(part 1 of 2)
# Autodesk Inventor assembly: 110033226_iam_02_造型房屋一
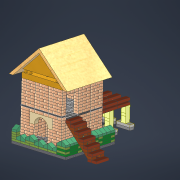
[picture p0: Inventor's stored thumbnail of the model, 180x180]
Saved by Autodesk Inventor 2022 (Build 260153000, 153)
## iProperties
Created: 2022-06-22
Part Number: 110033226_iam_02_造型房屋一
Document SubType Name: Assembly
Designer: User
Author: User
## Documents named in this file (14)
- D:\D-disk\pomelo\大一\下學期\機械設計製圖\1100332260_LEGOproj_沒有公主城堡\110033226_iam_02_造型房屋一.iam
- D:\D-disk\pomelo\大一\下學期\機械設計製圖\1100332260_LEGOproj_沒有公主城堡\110033226_ipt_05_房子底座.ipt
- D:\D-disk\pomelo\大一\下學期\機械設計製圖\1100332260_LEGOproj_沒有公主城堡\110033226_ipt_06_磚塊樺木(1x1).ipt
- D:\D-disk\pomelo\大一\下學期\機械設計製圖\1100332260_LEGOproj_沒有公主城堡\110033226_ipt_07_磚塊樺木(2x1).ipt
- D:\D-disk\pomelo\大一\下學期\機械設計製圖\1100332260_LEGOproj_沒有公主城堡\110033226_ipt_08_平滑面(3x1).ipt
- D:\D-disk\pomelo\大一\下學期\機械設計製圖\1100332260_LEGOproj_沒有公主城堡\110033226_ipt_09_窗戶圓拱.ipt
- D:\D-disk\pomelo\大一\下學期\機械設計製圖\1100332260_LEGOproj_沒有公主城堡\110033226_ipt_02_草地一.ipt
- D:\D-disk\pomelo\大一\下學期\機械設計製圖\1100332260_LEGOproj_沒有公主城堡\110033226_ipt_10_木板條.ipt
- D:\D-disk\pomelo\大一\下學期\機械設計製圖\1100332260_LEGOproj_沒有公主城堡\110033226_ipt_11_樓梯支架.ipt
- D:\D-disk\pomelo\大一\下學期\機械設計製圖\1100332260_LEGOproj_沒有公主城堡\110033226_ipt_12_平滑面(2x1).ipt
- D:\D-disk\pomelo\大一\下學期\機械設計製圖\1100332260_LEGOproj_沒有公主城堡\110033226_ipt_13_草地二.ipt
- D:\D-disk\pomelo\大一\下學期\機械設計製圖\1100332260_LEGOproj_沒有公主城堡\110033226_ipt_14_草地三.ipt
- D:\D-disk\pomelo\大一\下學期\機械設計製圖\1100332260_LEGOproj_沒有公主城堡\110033226_ipt_15_房子屋頂.ipt
- D:\D-disk\pomelo\大一\下學期\機械設計製圖\1100332260_LEGOproj_沒有公主城堡\110033226_ipt_24_直條(3x1).ipt
## Components (694 placed, 13 different names)
1. 110033226_ipt_05_房子底座:1 — 貼合:1, 貼合:2, 貼合:3, 貼合:4, 貼合:6, 貼合:8, 貼合:9, 貼合:10, 貼合:11, 貼合:12, 貼合:13, 貼合:14, 貼合:15, 貼合:16, 貼合:17, 貼合:18, 貼合:19, 貼合:20, 貼合:21, 貼合:22, 貼合:23, 貼合:24, 貼合:25, 貼合:26, 貼合:27, 貼合:28, 貼合:173, 貼合:292, 貼合:293, 貼合:294, 貼合:295, 貼合:296, 貼合:297, 貼合:298, 貼合:299, 貼合:300, 貼合:301, 貼合:302, 貼合:303, 貼合:310, 貼合:311, 貼合:312
2. 110033226_ipt_06_磚塊樺木(1x1):22 — 貼合:37, 貼合:38, 貼合:58, 貼合:59, 貼合:69
3. 110033226_ipt_07_磚塊樺木(2x1):23 — 貼合:34, 貼合:35, 貼合:36, 貼合:60, 貼合:61, 貼合:62
4. 110033226_ipt_06_磚塊樺木(1x1):24 — 貼合:41, 貼合:42, 貼合:68
5. 110033226_ipt_07_磚塊樺木(2x1):25 — 貼合:39, 貼合:40, 貼合:68
6. 110033226_ipt_08_平滑面(3x1):3 — 貼合:93, 貼合:94, 貼合:95
7. 110033226_ipt_09_窗戶圓拱:1 — 貼合:117, 貼合:118, 貼合:119, 貼合:152
8. 110033226_ipt_10_木板條:2 — 貼合:171, 貼合:172, 貼合:173, 貼合:174, 貼合:175, 貼合:176
9. 110033226_ipt_10_木板條:3 — 貼合:177, 貼合:178, 貼合:179
10. 110033226_ipt_10_木板條:4 — 貼合:182, 貼合:186, 貼合:187
11. 110033226_ipt_10_木板條:5 — 貼合:181, 貼合:184, 貼合:185
12. 110033226_ipt_10_木板條:6 — 貼合:183, 貼合:188, 貼合:189
13. 110033226_ipt_10_木板條:7 — 貼合:180, 貼合:190, 貼合:191
14. 110033226_ipt_07_磚塊樺木(2x1):234
15. 110033226_ipt_06_磚塊樺木(1x1):216
16. 110033226_ipt_07_磚塊樺木(2x1):233
17. 110033226_ipt_06_磚塊樺木(1x1):215
18. 110033226_ipt_06_磚塊樺木(1x1):239 — 貼合:246, 貼合:247, 貼合:248, 貼合:264
19. 110033226_ipt_07_磚塊樺木(2x1):257 — 貼合:240, 貼合:241, 貼合:242, 貼合:243, 貼合:244, 貼合:245, 貼合:262
20. 110033226_ipt_06_磚塊樺木(1x1):240 — 貼合:243, 貼合:244, 貼合:245, 貼合:246, 貼合:247, 貼合:248, 貼合:261, 貼合:263
21. 110033226_ipt_07_磚塊樺木(2x1):260 — 貼合:261, 貼合:262, 貼合:263, 貼合:266
22. 110033226_ipt_06_磚塊樺木(1x1):249 — 貼合:264, 貼合:265, 貼合:266
23. 110033226_ipt_06_磚塊樺木(1x1):272
24. 110033226_ipt_08_平滑面(3x1):34 — 貼合:286, 貼合:287, 貼合:288, 貼合:291
25. 110033226_ipt_08_平滑面(3x1):35 — 貼合:283, 貼合:284, 貼合:285
26. 110033226_ipt_12_平滑面(2x1):1 — 貼合:289, 貼合:290, 貼合:291
27. 110033226_ipt_14_草地三:2 — 貼合:307, 貼合:308, 貼合:309, 貼合:315, 貼合:320
28. 110033226_ipt_14_草地三:3 — 貼合:313, 貼合:314, 貼合:315
29. 110033226_ipt_14_草地三:4 — 貼合:319, 貼合:320, 貼合:321, 貼合:338
30. 110033226_ipt_13_草地二:20 — 貼合:331, 貼合:332, 貼合:333, 貼合:334, 貼合:335, 對稱:4, 貼合:369, 貼合:370, 貼合:396
31. 110033226_ipt_13_草地二:21 — 貼合:356, 貼合:357, 貼合:358, 貼合:361, 貼合:363, 貼合:364, 貼合:392, 貼合:393
32. 110033226_ipt_13_草地二:22 — 貼合:339, 貼合:340, 貼合:341, 貼合:343, 貼合:383, 貼合:384, 貼合:385, 貼合:386, 貼合:387
33. 110033226_ipt_13_草地二:23 — 貼合:353, 貼合:354, 貼合:355, 貼合:356, 貼合:357, 貼合:358
34. 110033226_ipt_14_草地三:5 — 貼合:336, 貼合:337, 貼合:338
35. 110033226_ipt_14_草地三:6 — 貼合:325, 貼合:326, 貼合:327, 貼合:329
36. 110033226_ipt_14_草地三:7 — 貼合:334, 貼合:335, 對稱:4, 貼合:368
37. 110033226_ipt_14_草地三:8 — 貼合:322, 貼合:323, 貼合:324, 貼合:367
38. 110033226_ipt_14_草地三:9 — 貼合:328, 貼合:329, 貼合:330
39. 110033226_ipt_14_草地三:10 — 貼合:344, 貼合:345, 貼合:346, 貼合:349
40. 110033226_ipt_14_草地三:11 — 貼合:350, 貼合:351, 貼合:352
41. 110033226_ipt_14_草地三:12 — 貼合:342, 貼合:343, 貼合:346
42. 110033226_ipt_14_草地三:13 — 貼合:347, 貼合:348, 貼合:349, 貼合:352
43. 110033226_ipt_14_草地三:14 — 貼合:361, 貼合:363, 貼合:364
44. 110033226_ipt_14_草地三:16 — 貼合:365, 貼合:366, 貼合:367, 貼合:390
45. 110033226_ipt_14_草地三:17 — 貼合:368, 貼合:369, 貼合:370
46. 110033226_ipt_14_草地三:42 — 貼合:383, 貼合:384, 貼合:385, 貼合:388
47. 110033226_ipt_14_草地三:43 — 貼合:386, 貼合:387, 貼合:388
48. 110033226_ipt_14_草地三:44 — 貼合:389, 貼合:390, 貼合:391
49. 110033226_ipt_14_草地三:45 — 貼合:397, 貼合:398, 貼合:399
50. 110033226_ipt_14_草地三:46 — 貼合:394, 貼合:395, 貼合:396, 貼合:398
51. 110033226_ipt_14_草地三:47 — 貼合:392, 貼合:393
52. 110033226_ipt_15_房子屋頂:1 — 貼合:400, 貼合:401, 貼合:402
53. 110033226_ipt_07_磚塊樺木(2x1):1 — 貼合:4, 貼合:8, 貼合:10, 貼合:29, 貼合:30, 貼合:31, 貼合:32
54. 110033226_ipt_06_磚塊樺木(1x1):1 — 貼合:6, 貼合:9, 貼合:33
55. 110033226_ipt_07_磚塊樺木(2x1):3
56. 110033226_ipt_06_磚塊樺木(1x1):3
57. 110033226_ipt_07_磚塊樺木(2x1):4
58. 110033226_ipt_06_磚塊樺木(1x1):4
59. 110033226_ipt_06_磚塊樺木(1x1):2 — 貼合:11, 貼合:13, 貼合:43, 貼合:45
60. 110033226_ipt_07_磚塊樺木(2x1):2 — 貼合:12, 貼合:14, 貼合:15, 貼合:44, 貼合:46, 貼合:47
61. 110033226_ipt_06_磚塊樺木(1x1):5
62. 110033226_ipt_07_磚塊樺木(2x1):5
63. 110033226_ipt_06_磚塊樺木(1x1):6
64. 110033226_ipt_07_磚塊樺木(2x1):6
65. 110033226_ipt_06_磚塊樺木(1x1):7
66. 110033226_ipt_07_磚塊樺木(2x1):7
67. 110033226_ipt_06_磚塊樺木(1x1):8
68. 110033226_ipt_07_磚塊樺木(2x1):8
69. 110033226_ipt_06_磚塊樺木(1x1):9
70. 110033226_ipt_07_磚塊樺木(2x1):9
71. 110033226_ipt_07_磚塊樺木(2x1):10 — 貼合:17, 貼合:18, 貼合:19, 貼合:49, 貼合:54, 貼合:55
72. 110033226_ipt_06_磚塊樺木(1x1):10 — 貼合:16, 貼合:20, 貼合:48, 貼合:50
73. 110033226_ipt_07_磚塊樺木(2x1):11
74. 110033226_ipt_06_磚塊樺木(1x1):11
75. 110033226_ipt_07_磚塊樺木(2x1):12
76. 110033226_ipt_06_磚塊樺木(1x1):12
77. 110033226_ipt_07_磚塊樺木(2x1):13
78. 110033226_ipt_06_磚塊樺木(1x1):13
79. 110033226_ipt_07_磚塊樺木(2x1):14
80. 110033226_ipt_06_磚塊樺木(1x1):14
81. 110033226_ipt_07_磚塊樺木(2x1):15
82. 110033226_ipt_06_磚塊樺木(1x1):15
83. 110033226_ipt_06_磚塊樺木(1x1):17 — 貼合:30, 貼合:31, 貼合:34, 貼合:35, 貼合:70
84. 110033226_ipt_07_磚塊樺木(2x1):18 — 貼合:29, 貼合:32, 貼合:33, 貼合:36, 貼合:37, 貼合:38, 貼合:70
85. 110033226_ipt_06_磚塊樺木(1x1):18 — 貼合:69, 貼合:95
86. 110033226_ipt_07_磚塊樺木(2x1):19 — 貼合:93, 貼合:94
87. 110033226_ipt_06_磚塊樺木(1x1):19 — 貼合:39, 貼合:40
88. 110033226_ipt_07_磚塊樺木(2x1):20 — 貼合:41, 貼合:42
89. 110033226_ipt_07_磚塊樺木(2x1):21 — 貼合:43, 貼合:45, 貼合:46, 貼合:53, 貼合:56, 貼合:57
90. 110033226_ipt_06_磚塊樺木(1x1):25 — 貼合:44, 貼合:47, 貼合:51, 貼合:52
91. 110033226_ipt_07_磚塊樺木(2x1):27
92. 110033226_ipt_06_磚塊樺木(1x1):26
93. 110033226_ipt_07_磚塊樺木(2x1):28
94. 110033226_ipt_06_磚塊樺木(1x1):27
95. 110033226_ipt_07_磚塊樺木(2x1):29
96. 110033226_ipt_06_磚塊樺木(1x1):28
97. 110033226_ipt_07_磚塊樺木(2x1):30
98. 110033226_ipt_06_磚塊樺木(1x1):29
99. 110033226_ipt_07_磚塊樺木(2x1):31
100. 110033226_ipt_06_磚塊樺木(1x1):30
101. 110033226_ipt_06_磚塊樺木(1x1):20 — 貼合:54, 貼合:55, 貼合:63, 貼合:64
102. 110033226_ipt_07_磚塊樺木(2x1):22 — 貼合:48, 貼合:49, 貼合:50, 貼合:65, 貼合:66, 貼合:67
103. 110033226_ipt_06_磚塊樺木(1x1):31
104. 110033226_ipt_07_磚塊樺木(2x1):32
105. 110033226_ipt_06_磚塊樺木(1x1):32
106. 110033226_ipt_07_磚塊樺木(2x1):33
107. 110033226_ipt_06_磚塊樺木(1x1):33
108. 110033226_ipt_07_磚塊樺木(2x1):34
109. 110033226_ipt_06_磚塊樺木(1x1):34
110. 110033226_ipt_07_磚塊樺木(2x1):35
111. 110033226_ipt_06_磚塊樺木(1x1):35
112. 110033226_ipt_07_磚塊樺木(2x1):36
113. 110033226_ipt_06_磚塊樺木(1x1):43 — 貼合:66, 貼合:67, 貼合:72, 貼合:77
114. 110033226_ipt_07_磚塊樺木(2x1):46 — 貼合:63, 貼合:64, 貼合:65, 貼合:72, 貼合:73, 貼合:74, 貼合:75, 貼合:76
115. 110033226_ipt_06_磚塊樺木(1x1):52
116. 110033226_ipt_07_磚塊樺木(2x1):53
117. 110033226_ipt_06_磚塊樺木(1x1):53
118. 110033226_ipt_07_磚塊樺木(2x1):54
119. 110033226_ipt_06_磚塊樺木(1x1):54
120. 110033226_ipt_07_磚塊樺木(2x1):55
121. 110033226_ipt_06_磚塊樺木(1x1):55
122. 110033226_ipt_07_磚塊樺木(2x1):56
123. 110033226_ipt_06_磚塊樺木(1x1):56
124. 110033226_ipt_07_磚塊樺木(2x1):57
125. 110033226_ipt_07_磚塊樺木(2x1):44 — 貼合:75, 貼合:76, 貼合:77, 貼合:78, 貼合:80, 貼合:82, 貼合:83
126. 110033226_ipt_06_磚塊樺木(1x1):42 — 貼合:73, 貼合:74, 貼合:78, 貼合:79, 貼合:81
127. 110033226_ipt_07_磚塊樺木(2x1):58
128. 110033226_ipt_06_磚塊樺木(1x1):57
129. 110033226_ipt_07_磚塊樺木(2x1):59
130. 110033226_ipt_06_磚塊樺木(1x1):58
131. 110033226_ipt_07_磚塊樺木(2x1):60
132. 110033226_ipt_06_磚塊樺木(1x1):59
133. 110033226_ipt_07_磚塊樺木(2x1):61
134. 110033226_ipt_06_磚塊樺木(1x1):60
135. 110033226_ipt_07_磚塊樺木(2x1):62
136. 110033226_ipt_06_磚塊樺木(1x1):61
137. 110033226_ipt_06_磚塊樺木(1x1):23 — 貼合:61, 貼合:62, 貼合:71
138. 110033226_ipt_07_磚塊樺木(2x1):26 — 貼合:58, 貼合:59, 貼合:60, 貼合:71
139. 110033226_ipt_06_磚塊樺木(1x1):62 — 貼合:87, 貼合:89
140. 110033226_ipt_07_磚塊樺木(2x1):63 — 貼合:88, 貼合:96, 貼合:97
141. 110033226_ipt_07_磚塊樺木(2x1):52 — 貼合:87, 貼合:88, 貼合:89, 貼合:98, 貼合:99, 貼合:101, 貼合:105, 貼合:106
142. 110033226_ipt_06_磚塊樺木(1x1):45 — 貼合:96, 貼合:97, 貼合:98, 貼合:100
143. 110033226_ipt_06_磚塊樺木(1x1):47 — 貼合:105, 貼合:106, 貼合:107, 貼合:113
144. 110033226_ipt_07_磚塊樺木(2x1):51 — 貼合:99, 貼合:100, 貼合:101, 貼合:104, 貼合:107, 貼合:111, 貼合:112, 貼合:114, 貼合:115
145. 110033226_ipt_07_磚塊樺木(2x1):47 — 貼合:111, 貼合:112, 貼合:113, 貼合:116, 貼合:117, 貼合:134
146. 110033226_ipt_06_磚塊樺木(1x1):46 — 貼合:114, 貼合:115, 貼合:116, 貼合:132, 貼合:133
147. 110033226_ipt_07_磚塊樺木(2x1):64
148. 110033226_ipt_06_磚塊樺木(1x1):63
149. 110033226_ipt_06_磚塊樺木(1x1):64
150. 110033226_ipt_07_磚塊樺木(2x1):65
151. 110033226_ipt_07_磚塊樺木(2x1):66
152. 110033226_ipt_06_磚塊樺木(1x1):65 — 貼合:118, 貼合:119
153. 110033226_ipt_07_磚塊樺木(2x1):75 — 貼合:132, 貼合:133, 貼合:134, 貼合:141, 貼合:142, 貼合:143
154. 110033226_ipt_07_磚塊樺木(2x1):78 — 貼合:141, 貼合:142, 貼合:143, 貼合:144, 貼合:145, 貼合:146
155. 110033226_ipt_07_磚塊樺木(2x1):73 — 貼合:144, 貼合:145, 貼合:146, 貼合:147, 貼合:148, 貼合:149
156. 110033226_ipt_07_磚塊樺木(2x1):72 — 貼合:147, 貼合:148, 貼合:149, 貼合:150, 貼合:151, 貼合:153
157. 110033226_ipt_07_磚塊樺木(2x1):80
158. 110033226_ipt_07_磚塊樺木(2x1):81
159. 110033226_ipt_07_磚塊樺木(2x1):82
160. 110033226_ipt_07_磚塊樺木(2x1):83
161. 110033226_ipt_07_磚塊樺木(2x1):74 — 貼合:152, 貼合:153, 貼合:154, 貼合:155, 貼合:157
162. 110033226_ipt_06_磚塊樺木(1x1):71 — 貼合:150, 貼合:151, 貼合:154, 貼合:156
163. 110033226_ipt_07_磚塊樺木(2x1):84
164. 110033226_ipt_06_磚塊樺木(1x1):77
165. 110033226_ipt_07_磚塊樺木(2x1):85
166. 110033226_ipt_06_磚塊樺木(1x1):78
167. 110033226_ipt_08_平滑面(3x1):2 — 貼合:155, 貼合:156, 貼合:157, 貼合:211, 貼合:212, 貼合:213, 貼合:214
168. 110033226_ipt_08_平滑面(3x1):6 — 貼合:216
169. 110033226_ipt_08_平滑面(3x1):7
170. 110033226_ipt_07_磚塊樺木(2x1):17 — 貼合:23, 貼合:27, 貼合:28, 貼合:289, 貼合:290
171. 110033226_ipt_06_磚塊樺木(1x1):16 — 貼合:22, 貼合:24, 貼合:192, 貼合:288
172. 110033226_ipt_07_磚塊樺木(2x1):16 — 貼合:21, 貼合:25, 貼合:26, 貼合:192, 貼合:286, 貼合:287
173. 110033226_ipt_07_磚塊樺木(2x1):181 — 貼合:403, 貼合:404, 貼合:405
174. 110033226_ipt_06_磚塊樺木(1x1):168
175. 110033226_ipt_07_磚塊樺木(2x1):182
176. 110033226_ipt_07_磚塊樺木(2x1):183
177. 110033226_ipt_06_磚塊樺木(1x1):169
178. 110033226_ipt_07_磚塊樺木(2x1):184
179. 110033226_ipt_07_磚塊樺木(2x1):185
180. 110033226_ipt_06_磚塊樺木(1x1):170
181. 110033226_ipt_07_磚塊樺木(2x1):186
182. 110033226_ipt_07_磚塊樺木(2x1):187 — 貼合:194
183. 110033226_ipt_06_磚塊樺木(1x1):171 — 貼合:193, 貼合:195
184. 110033226_ipt_07_磚塊樺木(2x1):188 — 貼合:196, 貼合:197
185. 110033226_ipt_08_平滑面(3x1):1 — 貼合:193, 貼合:194, 貼合:195, 貼合:268, 貼合:270, 貼合:271
186. 110033226_ipt_08_平滑面(3x1):19
187. 110033226_ipt_08_平滑面(3x1):20
188. 110033226_ipt_08_平滑面(3x1):21
189. 110033226_ipt_08_平滑面(3x1):22
190. 110033226_ipt_08_平滑面(3x1):23
191. 110033226_ipt_08_平滑面(3x1):24
192. 110033226_ipt_08_平滑面(3x1):25
193. 110033226_ipt_08_平滑面(3x1):26
194. 110033226_ipt_08_平滑面(3x1):4 — 貼合:196, 貼合:197, 貼合:198
195. 110033226_ipt_08_平滑面(3x1):27
196. 110033226_ipt_08_平滑面(3x1):28
197. 110033226_ipt_08_平滑面(3x1):29
198. 110033226_ipt_08_平滑面(3x1):30
199. 110033226_ipt_08_平滑面(3x1):31
200. 110033226_ipt_07_磚塊樺木(2x1):76 — 貼合:205, 貼合:206, 貼合:207, 貼合:210
201. 110033226_ipt_06_磚塊樺木(1x1):73 — 貼合:208, 貼合:209, 貼合:210
202. 110033226_ipt_06_磚塊樺木(1x1):66 — 貼合:199, 貼合:200, 貼合:201, 貼合:203, 貼合:205, 貼合:206
203. 110033226_ipt_07_磚塊樺木(2x1):69 — 貼合:202, 貼合:203, 貼合:204, 貼合:207, 貼合:208, 貼合:209
204. 110033226_ipt_07_磚塊樺木(2x1):189
205. 110033226_ipt_06_磚塊樺木(1x1):172
206. 110033226_ipt_06_磚塊樺木(1x1):173
207. 110033226_ipt_07_磚塊樺木(2x1):190 — 貼合:269
208. 110033226_ipt_07_磚塊樺木(2x1):191
209. 110033226_ipt_06_磚塊樺木(1x1):174
210. 110033226_ipt_06_磚塊樺木(1x1):175
211. 110033226_ipt_07_磚塊樺木(2x1):192
212. 110033226_ipt_07_磚塊樺木(2x1):193
213. 110033226_ipt_06_磚塊樺木(1x1):176
214. 110033226_ipt_06_磚塊樺木(1x1):177
215. 110033226_ipt_07_磚塊樺木(2x1):194
216. 110033226_ipt_07_磚塊樺木(2x1):195
217. 110033226_ipt_06_磚塊樺木(1x1):178
218. 110033226_ipt_06_磚塊樺木(1x1):179
219. 110033226_ipt_07_磚塊樺木(2x1):196
220. 110033226_ipt_07_磚塊樺木(2x1):197
221. 110033226_ipt_06_磚塊樺木(1x1):180
222. 110033226_ipt_06_磚塊樺木(1x1):181
223. 110033226_ipt_07_磚塊樺木(2x1):198
224. 110033226_ipt_07_磚塊樺木(2x1):199
225. 110033226_ipt_06_磚塊樺木(1x1):182
226. 110033226_ipt_06_磚塊樺木(1x1):183
227. 110033226_ipt_07_磚塊樺木(2x1):200
228. 110033226_ipt_07_磚塊樺木(2x1):201
229. 110033226_ipt_06_磚塊樺木(1x1):184
230. 110033226_ipt_06_磚塊樺木(1x1):185
231. 110033226_ipt_07_磚塊樺木(2x1):202
232. 110033226_ipt_07_磚塊樺木(2x1):203 — 貼合:265
233. 110033226_ipt_06_磚塊樺木(1x1):186
234. 110033226_ipt_06_磚塊樺木(1x1):187
235. 110033226_ipt_07_磚塊樺木(2x1):204
236. 110033226_ipt_07_磚塊樺木(2x1):205
237. 110033226_ipt_06_磚塊樺木(1x1):188
238. 110033226_ipt_06_磚塊樺木(1x1):189
239. 110033226_ipt_07_磚塊樺木(2x1):206
240. 110033226_ipt_07_磚塊樺木(2x1):68 — 貼合:211, 貼合:212, 貼合:213, 貼合:215, 貼合:228, 貼合:230, 貼合:231, 貼合:232
241. 110033226_ipt_06_磚塊樺木(1x1):75 — 貼合:214, 貼合:215, 貼合:216, 貼合:229
242. 110033226_ipt_07_磚塊樺木(2x1):207
243. 110033226_ipt_06_磚塊樺木(1x1):190
244. 110033226_ipt_07_磚塊樺木(2x1):208
245. 110033226_ipt_06_磚塊樺木(1x1):191
246. 110033226_ipt_06_磚塊樺木(1x1):68 — 貼合:217, 貼合:218, 貼合:219, 貼合:222, 貼合:223, 貼合:224
247. 110033226_ipt_07_磚塊樺木(2x1):210 — 貼合:223, 貼合:224, 貼合:225, 貼合:226
248. 110033226_ipt_06_磚塊樺木(1x1):192 — 對稱:2, 貼合:226, 貼合:227
249. 110033226_ipt_07_磚塊樺木(2x1):209 — 貼合:220, 貼合:221, 貼合:222, 貼合:225, 對稱:2, 貼合:227
250. 110033226_ipt_06_磚塊樺木(1x1):193
251. 110033226_ipt_07_磚塊樺木(2x1):211
252. 110033226_ipt_06_磚塊樺木(1x1):194
253. 110033226_ipt_07_磚塊樺木(2x1):212
254. 110033226_ipt_06_磚塊樺木(1x1):195
255. 110033226_ipt_07_磚塊樺木(2x1):213
256. 110033226_ipt_06_磚塊樺木(1x1):196
257. 110033226_ipt_07_磚塊樺木(2x1):214
258. 110033226_ipt_06_磚塊樺木(1x1):197
259. 110033226_ipt_07_磚塊樺木(2x1):215
260. 110033226_ipt_06_磚塊樺木(1x1):198
261. 110033226_ipt_07_磚塊樺木(2x1):216
262. 110033226_ipt_06_磚塊樺木(1x1):199
263. 110033226_ipt_07_磚塊樺木(2x1):217
264. 110033226_ipt_06_磚塊樺木(1x1):200
265. 110033226_ipt_07_磚塊樺木(2x1):218
266. 110033226_ipt_06_磚塊樺木(1x1):201
267. 110033226_ipt_07_磚塊樺木(2x1):219
268. 110033226_ipt_06_磚塊樺木(1x1):202
269. 110033226_ipt_07_磚塊樺木(2x1):220
270. 110033226_ipt_06_磚塊樺木(1x1):203
271. 110033226_ipt_07_磚塊樺木(2x1):221 — 貼合:283, 貼合:285
272. 110033226_ipt_06_磚塊樺木(1x1):204 — 貼合:284
273. 110033226_ipt_07_磚塊樺木(2x1):222
274. 110033226_ipt_06_磚塊樺木(1x1):209
275. 110033226_ipt_07_磚塊樺木(2x1):227
276. 110033226_ipt_06_磚塊樺木(1x1):210
277. 110033226_ipt_07_磚塊樺木(2x1):228
278. 110033226_ipt_06_磚塊樺木(1x1):211
279. 110033226_ipt_07_磚塊樺木(2x1):229
280. 110033226_ipt_06_磚塊樺木(1x1):212
281. 110033226_ipt_07_磚塊樺木(2x1):230
282. 110033226_ipt_06_磚塊樺木(1x1):213
283. 110033226_ipt_07_磚塊樺木(2x1):231
284. 110033226_ipt_06_磚塊樺木(1x1):214
285. 110033226_ipt_07_磚塊樺木(2x1):232
286. 110033226_ipt_06_磚塊樺木(1x1):217
287. 110033226_ipt_07_磚塊樺木(2x1):235
288. 110033226_ipt_06_磚塊樺木(1x1):218
289. 110033226_ipt_07_磚塊樺木(2x1):236
290. 110033226_ipt_06_磚塊樺木(1x1):219
291. 110033226_ipt_07_磚塊樺木(2x1):237
292. 110033226_ipt_06_磚塊樺木(1x1):220
293. 110033226_ipt_07_磚塊樺木(2x1):238
294. 110033226_ipt_06_磚塊樺木(1x1):222 — 貼合:237, 貼合:238, 貼合:239
295. 110033226_ipt_07_磚塊樺木(2x1):239 — 貼合:228, 貼合:229, 貼合:230, 貼合:233, 貼合:236, 貼合:237, 貼合:238
296. 110033226_ipt_06_磚塊樺木(1x1):221 — 貼合:231, 貼合:232, 貼合:233, 貼合:234, 貼合:235
297. 110033226_ipt_07_磚塊樺木(2x1):240 — 貼合:234, 貼合:235, 貼合:236, 貼合:239
298. 110033226_ipt_06_磚塊樺木(1x1):223
299. 110033226_ipt_07_磚塊樺木(2x1):241
300. 110033226_ipt_06_磚塊樺木(1x1):224
301. 110033226_ipt_07_磚塊樺木(2x1):242
302. 110033226_ipt_06_磚塊樺木(1x1):225
303. 110033226_ipt_07_磚塊樺木(2x1):243
304. 110033226_ipt_06_磚塊樺木(1x1):226
305. 110033226_ipt_07_磚塊樺木(2x1):244 — 貼合:240, 貼合:241, 貼合:242
306. 110033226_ipt_06_磚塊樺木(1x1):227
307. 110033226_ipt_07_磚塊樺木(2x1):245
308. 110033226_ipt_06_磚塊樺木(1x1):228
309. 110033226_ipt_07_磚塊樺木(2x1):246
310. 110033226_ipt_06_磚塊樺木(1x1):229
311. 110033226_ipt_07_磚塊樺木(2x1):247
312. 110033226_ipt_06_磚塊樺木(1x1):230
313. 110033226_ipt_07_磚塊樺木(2x1):248
314. 110033226_ipt_06_磚塊樺木(1x1):231
315. 110033226_ipt_07_磚塊樺木(2x1):249
316. 110033226_ipt_06_磚塊樺木(1x1):232
317. 110033226_ipt_07_磚塊樺木(2x1):250
318. 110033226_ipt_06_磚塊樺木(1x1):233
319. 110033226_ipt_07_磚塊樺木(2x1):251
320. 110033226_ipt_06_磚塊樺木(1x1):234
321. 110033226_ipt_07_磚塊樺木(2x1):252
322. 110033226_ipt_06_磚塊樺木(1x1):235
323. 110033226_ipt_07_磚塊樺木(2x1):253
324. 110033226_ipt_06_磚塊樺木(1x1):236
325. 110033226_ipt_07_磚塊樺木(2x1):254
326. 110033226_ipt_06_磚塊樺木(1x1):237 — 貼合:249, 貼合:250
327. 110033226_ipt_07_磚塊樺木(2x1):255
328. 110033226_ipt_06_磚塊樺木(1x1):238
329. 110033226_ipt_07_磚塊樺木(2x1):256 — 貼合:251, 貼合:252, 貼合:253
330. 110033226_ipt_07_磚塊樺木(2x1):259 — 貼合:258, 貼合:259, 貼合:260
331. 110033226_ipt_06_磚塊樺木(1x1):242 — 貼合:255, 貼合:256, 貼合:257, 貼合:402
332. 110033226_ipt_07_磚塊樺木(2x1):258 — 貼合:249, 貼合:250, 貼合:251, 貼合:254, 貼合:255, 貼合:256, 貼合:257, 貼合:258
333. 110033226_ipt_06_磚塊樺木(1x1):241 — 貼合:252, 貼合:253, 貼合:254, 貼合:259, 貼合:260
334. 110033226_ipt_07_磚塊樺木(2x1):261
335. 110033226_ipt_06_磚塊樺木(1x1):243
336. 110033226_ipt_07_磚塊樺木(2x1):262
337. 110033226_ipt_06_磚塊樺木(1x1):244
338. 110033226_ipt_07_磚塊樺木(2x1):263 — 貼合:400, 貼合:401
339. 110033226_ipt_06_磚塊樺木(1x1):245
340. 110033226_ipt_07_磚塊樺木(2x1):264
341. 110033226_ipt_06_磚塊樺木(1x1):246
342. 110033226_ipt_07_磚塊樺木(2x1):265 — 貼合:267, 貼合:268, 貼合:269, 貼合:272, 貼合:273, 貼合:275, 貼合:276
343. 110033226_ipt_07_磚塊樺木(2x1):266 — 對稱:3, 貼合:273, 貼合:274, 貼合:277
344. 110033226_ipt_06_磚塊樺木(1x1):248 — 貼合:270, 貼合:271, 貼合:272, 對稱:3, 貼合:274
345. 110033226_ipt_06_磚塊樺木(1x1):247 — 貼合:275, 貼合:276, 貼合:277
346. 110033226_ipt_07_磚塊樺木(2x1):268
347. 110033226_ipt_07_磚塊樺木(2x1):269 — 貼合:281, 貼合:282
348. 110033226_ipt_06_磚塊樺木(1x1):250
349. 110033226_ipt_06_磚塊樺木(1x1):251 — 貼合:280
350. 110033226_ipt_07_磚塊樺木(2x1):274
351. 110033226_ipt_07_磚塊樺木(2x1):275
352. 110033226_ipt_06_磚塊樺木(1x1):256
353. 110033226_ipt_06_磚塊樺木(1x1):257
354. 110033226_ipt_07_磚塊樺木(2x1):276
355. 110033226_ipt_07_磚塊樺木(2x1):277
356. 110033226_ipt_06_磚塊樺木(1x1):258 — 貼合:279
357. 110033226_ipt_06_磚塊樺木(1x1):259
358. 110033226_ipt_07_磚塊樺木(2x1):278
359. 110033226_ipt_07_磚塊樺木(2x1):279
360. 110033226_ipt_06_磚塊樺木(1x1):260
361. 110033226_ipt_06_磚塊樺木(1x1):261
362. 110033226_ipt_07_磚塊樺木(2x1):284
363. 110033226_ipt_07_磚塊樺木(2x1):285
364. 110033226_ipt_06_磚塊樺木(1x1):266
365. 110033226_ipt_06_磚塊樺木(1x1):267
366. 110033226_ipt_06_磚塊樺木(1x1):268 — 貼合:278, 貼合:279
367. 110033226_ipt_06_磚塊樺木(1x1):269
368. 110033226_ipt_06_磚塊樺木(1x1):270
369. 110033226_ipt_06_磚塊樺木(1x1):271
370. 110033226_ipt_06_磚塊樺木(1x1):273
371. 110033226_ipt_06_磚塊樺木(1x1):274
372. 110033226_ipt_06_磚塊樺木(1x1):275
373. 110033226_ipt_06_磚塊樺木(1x1):276
374. 110033226_ipt_06_磚塊樺木(1x1):277
375. 110033226_ipt_08_平滑面(3x1):33 — 貼合:280, 貼合:281, 貼合:282
376. 110033226_ipt_08_平滑面(3x1):36
377. 110033226_ipt_13_草地二:1 — 貼合:292, 貼合:293, 貼合:294, 貼合:325
378. 110033226_ipt_13_草地二:4 — 貼合:326, 貼合:328, 貼合:330, 貼合:331, 貼合:332
379. 110033226_ipt_13_草地二:5 — 貼合:333, 貼合:394, 貼合:395, 貼合:399
380. 110033226_ipt_13_草地二:6 — 貼合:389, 貼合:391, 貼合:397
381. 110033226_ipt_13_草地二:7 — 貼合:322, 貼合:323, 貼合:365, 貼合:366
382. 110033226_ipt_13_草地二:2 — 貼合:295, 貼合:296, 貼合:297
383. 110033226_ipt_13_草地二:8
384. 110033226_ipt_13_草地二:9
385. 110033226_ipt_13_草地二:10 — 貼合:316, 貼合:318
386. 110033226_ipt_13_草地二:11 — 貼合:307, 貼合:308, 貼合:309, 貼合:317
387. 110033226_ipt_13_草地二:14 — 貼合:310, 貼合:311, 貼合:312, 貼合:313, 貼合:314
388. 110033226_ipt_13_草地二:15
389. 110033226_ipt_13_草地二:16
390. 110033226_ipt_13_草地二:17
391. 110033226_ipt_13_草地二:18
392. 110033226_ipt_13_草地二:19 — 貼合:316, 貼合:317, 貼合:318, 貼合:319, 貼合:321, 貼合:336, 貼合:337
393. 110033226_ipt_13_草地二:24 — 貼合:339, 貼合:340, 貼合:341
394. 110033226_ipt_13_草地二:25 — 貼合:342, 貼合:344, 貼合:345
395. 110033226_ipt_13_草地二:26 — 貼合:347, 貼合:348, 貼合:350, 貼合:351
396. 110033226_ipt_13_草地二:27 — 貼合:327, 貼合:353, 貼合:354, 貼合:355
397. 110033226_ipt_14_草地三:19 — 貼合:380, 貼合:381, 貼合:382
398. 110033226_ipt_14_草地三:18 — 貼合:377, 貼合:378, 貼合:379
399. 110033226_ipt_14_草地三:20
400. 110033226_ipt_14_草地三:21
401. 110033226_ipt_14_草地三:22
402. 110033226_ipt_14_草地三:23
403. 110033226_ipt_14_草地三:24
404. 110033226_ipt_14_草地三:25
405. 110033226_ipt_14_草地三:26
406. 110033226_ipt_14_草地三:27
407. 110033226_ipt_14_草地三:28
408. 110033226_ipt_14_草地三:29
409. 110033226_ipt_14_草地三:30
410. 110033226_ipt_14_草地三:31
411. 110033226_ipt_14_草地三:32
412. 110033226_ipt_14_草地三:33
413. 110033226_ipt_14_草地三:34
414. 110033226_ipt_14_草地三:35
415. 110033226_ipt_14_草地三:36
416. 110033226_ipt_14_草地三:37
417. 110033226_ipt_14_草地三:38
418. 110033226_ipt_14_草地三:39
419. 110033226_ipt_14_草地三:40
420. 110033226_ipt_14_草地三:41
421. 110033226_ipt_08_平滑面(3x1):37 — 貼合:411, 貼合:412, 貼合:413
422. 110033226_ipt_08_平滑面(3x1):40
423. 110033226_ipt_08_平滑面(3x1):41
424. 110033226_ipt_08_平滑面(3x1):42
425. 110033226_ipt_24_直條(3x1):3 — 貼合:407, 貼合:414
426. 110033226_ipt_24_直條(3x1):2 — 貼合:406, 貼合:409, 貼合:410, 貼合:418
427. 110033226_ipt_24_直條(3x1):4 — 貼合:416
428. 110033226_ipt_24_直條(3x1):5 — 貼合:417
429. 110033226_ipt_10_木板條:31 — 貼合:419, 貼合:420
430. 110033226_ipt_10_木板條:32
431. 110033226_ipt_10_木板條:33
432. 110033226_ipt_10_木板條:34
433. 110033226_ipt_10_木板條:35 — 貼合:421, 貼合:422, 貼合:423
434. 110033226_ipt_10_木板條:36
435. 110033226_ipt_06_磚塊樺木(1x1):44 — 貼合:82, 貼合:83, 貼合:86
436. 110033226_ipt_07_磚塊樺木(2x1):43 — 貼合:79, 貼合:80, 貼合:81, 貼合:84, 貼合:85, 貼合:102, 貼合:103
437. 110033226_ipt_06_磚塊樺木(1x1):51 — 貼合:102, 貼合:103, 貼合:104, 貼合:120, 貼合:121
438. 110033226_ipt_07_磚塊樺木(2x1):49 — 貼合:120, 貼合:121, 貼合:122, 貼合:125, 貼合:127, 貼合:129, 貼合:131
439. 110033226_ipt_06_磚塊樺木(1x1):48 — 貼合:123, 貼合:124, 貼合:125, 貼合:126, 貼合:128
440. 110033226_ipt_07_磚塊樺木(2x1):45 — 貼合:84, 貼合:85, 貼合:86, 貼合:122, 貼合:123, 貼合:124
441. 110033226_ipt_06_磚塊樺木(1x1):74 — 貼合:129, 貼合:130, 貼合:131, 貼合:135, 貼合:136
442. 110033226_ipt_07_磚塊樺木(2x1):79 — 貼合:135, 貼合:136, 貼合:137, 貼合:140, 貼合:158, 貼合:160, 貼合:161
443. 110033226_ipt_06_磚塊樺木(1x1):76 — 貼合:138, 貼合:139, 貼合:140, 對稱:1, 貼合:159
444. 110033226_ipt_07_磚塊樺木(2x1):70 — 貼合:126, 貼合:127, 貼合:128, 貼合:130, 貼合:137, 貼合:138, 貼合:139
445. 110033226_ipt_07_磚塊樺木(2x1):67 — 對稱:1, 貼合:158, 貼合:159, 角度:1, 貼合:163, 貼合:165, 貼合:166
446. 110033226_ipt_06_磚塊樺木(1x1):70 — 貼合:165, 貼合:166, 貼合:167, 貼合:168, 貼合:170
447. 110033226_ipt_07_磚塊樺木(2x1):71 — 貼合:162, 貼合:163, 貼合:164, 貼合:167, 貼合:169, 貼合:171
448. 110033226_ipt_06_磚塊樺木(1x1):69 — 貼合:160, 貼合:161, 角度:1, 貼合:162, 貼合:164
449. 110033226_ipt_08_平滑面(3x1):5 — 貼合:168, 貼合:169, 貼合:170, 貼合:172
450. 110033226_ipt_06_磚塊樺木(1x1):79
451. 110033226_ipt_07_磚塊樺木(2x1):86
452. 110033226_ipt_06_磚塊樺木(1x1):80
453. 110033226_ipt_07_磚塊樺木(2x1):87
454. 110033226_ipt_06_磚塊樺木(1x1):81
455. 110033226_ipt_07_磚塊樺木(2x1):88
456. 110033226_ipt_06_磚塊樺木(1x1):82
457. 110033226_ipt_07_磚塊樺木(2x1):89
458. 110033226_ipt_06_磚塊樺木(1x1):83
459. 110033226_ipt_07_磚塊樺木(2x1):90
460. 110033226_ipt_07_磚塊樺木(2x1):91
461. 110033226_ipt_06_磚塊樺木(1x1):84
462. 110033226_ipt_07_磚塊樺木(2x1):92
463. 110033226_ipt_06_磚塊樺木(1x1):85
464. 110033226_ipt_08_平滑面(3x1):8
465. 110033226_ipt_06_磚塊樺木(1x1):86
466. 110033226_ipt_07_磚塊樺木(2x1):93
467. 110033226_ipt_06_磚塊樺木(1x1):87
468. 110033226_ipt_07_磚塊樺木(2x1):94
469. 110033226_ipt_06_磚塊樺木(1x1):88
470. 110033226_ipt_07_磚塊樺木(2x1):95
471. 110033226_ipt_06_磚塊樺木(1x1):89
472. 110033226_ipt_07_磚塊樺木(2x1):96
473. 110033226_ipt_06_磚塊樺木(1x1):90
474. 110033226_ipt_07_磚塊樺木(2x1):97
475. 110033226_ipt_07_磚塊樺木(2x1):98
476. 110033226_ipt_06_磚塊樺木(1x1):91
477. 110033226_ipt_07_磚塊樺木(2x1):99
478. 110033226_ipt_06_磚塊樺木(1x1):92
479. 110033226_ipt_08_平滑面(3x1):9 — 貼合:199, 貼合:200, 貼合:201, 貼合:202
480. 110033226_ipt_06_磚塊樺木(1x1):93
481. 110033226_ipt_07_磚塊樺木(2x1):100
482. 110033226_ipt_06_磚塊樺木(1x1):94
483. 110033226_ipt_07_磚塊樺木(2x1):101
484. 110033226_ipt_06_磚塊樺木(1x1):95
485. 110033226_ipt_07_磚塊樺木(2x1):102
486. 110033226_ipt_06_磚塊樺木(1x1):96
487. 110033226_ipt_07_磚塊樺木(2x1):103
488. 110033226_ipt_06_磚塊樺木(1x1):97
489. 110033226_ipt_07_磚塊樺木(2x1):104
490. 110033226_ipt_07_磚塊樺木(2x1):105
491. 110033226_ipt_06_磚塊樺木(1x1):98
492. 110033226_ipt_07_磚塊樺木(2x1):106
493. 110033226_ipt_06_磚塊樺木(1x1):99
494. 110033226_ipt_08_平滑面(3x1):10
495. 110033226_ipt_06_磚塊樺木(1x1):100
496. 110033226_ipt_07_磚塊樺木(2x1):107
497. 110033226_ipt_06_磚塊樺木(1x1):101
498. 110033226_ipt_07_磚塊樺木(2x1):108
499. 110033226_ipt_06_磚塊樺木(1x1):102
500. 110033226_ipt_07_磚塊樺木(2x1):109
501. 110033226_ipt_06_磚塊樺木(1x1):103
502. 110033226_ipt_07_磚塊樺木(2x1):110
503. 110033226_ipt_06_磚塊樺木(1x1):104
504. 110033226_ipt_07_磚塊樺木(2x1):111
505. 110033226_ipt_07_磚塊樺木(2x1):112
506. 110033226_ipt_06_磚塊樺木(1x1):105
507. 110033226_ipt_07_磚塊樺木(2x1):113
508. 110033226_ipt_06_磚塊樺木(1x1):106
509. 110033226_ipt_08_平滑面(3x1):11 — 貼合:204
510. 110033226_ipt_06_磚塊樺木(1x1):107
511. 110033226_ipt_07_磚塊樺木(2x1):114
512. 110033226_ipt_06_磚塊樺木(1x1):108
513. 110033226_ipt_07_磚塊樺木(2x1):115
514. 110033226_ipt_06_磚塊樺木(1x1):109
515. 110033226_ipt_07_磚塊樺木(2x1):116
516. 110033226_ipt_06_磚塊樺木(1x1):110
517. 110033226_ipt_07_磚塊樺木(2x1):117
518. 110033226_ipt_06_磚塊樺木(1x1):111
519. 110033226_ipt_07_磚塊樺木(2x1):118
520. 110033226_ipt_07_磚塊樺木(2x1):119
521. 110033226_ipt_06_磚塊樺木(1x1):112
522. 110033226_ipt_07_磚塊樺木(2x1):120
523. 110033226_ipt_06_磚塊樺木(1x1):113
524. 110033226_ipt_08_平滑面(3x1):12 — 貼合:267
525. 110033226_ipt_06_磚塊樺木(1x1):114
526. 110033226_ipt_07_磚塊樺木(2x1):121
527. 110033226_ipt_06_磚塊樺木(1x1):115
528. 110033226_ipt_07_磚塊樺木(2x1):122
529. 110033226_ipt_06_磚塊樺木(1x1):116
530. 110033226_ipt_07_磚塊樺木(2x1):123
531. 110033226_ipt_06_磚塊樺木(1x1):117
532. 110033226_ipt_07_磚塊樺木(2x1):124
533. 110033226_ipt_06_磚塊樺木(1x1):118
534. 110033226_ipt_07_磚塊樺木(2x1):125
535. 110033226_ipt_07_磚塊樺木(2x1):126
536. 110033226_ipt_06_磚塊樺木(1x1):119
537. 110033226_ipt_07_磚塊樺木(2x1):127
538. 110033226_ipt_06_磚塊樺木(1x1):120
539. 110033226_ipt_08_平滑面(3x1):13
540. 110033226_ipt_06_磚塊樺木(1x1):121
541. 110033226_ipt_07_磚塊樺木(2x1):128
542. 110033226_ipt_06_磚塊樺木(1x1):122
543. 110033226_ipt_07_磚塊樺木(2x1):129
544. 110033226_ipt_06_磚塊樺木(1x1):123
545. 110033226_ipt_07_磚塊樺木(2x1):130
546. 110033226_ipt_06_磚塊樺木(1x1):124
547. 110033226_ipt_07_磚塊樺木(2x1):131
548. 110033226_ipt_06_磚塊樺木(1x1):125
549. 110033226_ipt_07_磚塊樺木(2x1):132
550. 110033226_ipt_07_磚塊樺木(2x1):133
551. 110033226_ipt_06_磚塊樺木(1x1):126
552. 110033226_ipt_07_磚塊樺木(2x1):134
553. 110033226_ipt_06_磚塊樺木(1x1):127
554. 110033226_ipt_08_平滑面(3x1):14
555. 110033226_ipt_06_磚塊樺木(1x1):128
556. 110033226_ipt_07_磚塊樺木(2x1):135
557. 110033226_ipt_06_磚塊樺木(1x1):129
558. 110033226_ipt_07_磚塊樺木(2x1):136
559. 110033226_ipt_06_磚塊樺木(1x1):130
560. 110033226_ipt_07_磚塊樺木(2x1):137
561. 110033226_ipt_06_磚塊樺木(1x1):131
562. 110033226_ipt_07_磚塊樺木(2x1):138
563. 110033226_ipt_06_磚塊樺木(1x1):132
564. 110033226_ipt_07_磚塊樺木(2x1):139
565. 110033226_ipt_07_磚塊樺木(2x1):140
566. 110033226_ipt_06_磚塊樺木(1x1):133
567. 110033226_ipt_07_磚塊樺木(2x1):141
568. 110033226_ipt_06_磚塊樺木(1x1):134
569. 110033226_ipt_08_平滑面(3x1):15
570. 110033226_ipt_06_磚塊樺木(1x1):135
571. 110033226_ipt_07_磚塊樺木(2x1):142
572. 110033226_ipt_06_磚塊樺木(1x1):136
573. 110033226_ipt_07_磚塊樺木(2x1):143
574. 110033226_ipt_06_磚塊樺木(1x1):137
575. 110033226_ipt_07_磚塊樺木(2x1):144
576. 110033226_ipt_06_磚塊樺木(1x1):138
577. 110033226_ipt_07_磚塊樺木(2x1):145
578. 110033226_ipt_06_磚塊樺木(1x1):139
579. 110033226_ipt_07_磚塊樺木(2x1):146
580. 110033226_ipt_07_磚塊樺木(2x1):147
581. 110033226_ipt_06_磚塊樺木(1x1):140
582. 110033226_ipt_07_磚塊樺木(2x1):148
583. 110033226_ipt_06_磚塊樺木(1x1):141
584. 110033226_ipt_08_平滑面(3x1):16
585. 110033226_ipt_06_磚塊樺木(1x1):142
586. 110033226_ipt_07_磚塊樺木(2x1):149
587. 110033226_ipt_06_磚塊樺木(1x1):143
588. 110033226_ipt_07_磚塊樺木(2x1):150
589. 110033226_ipt_06_磚塊樺木(1x1):144
590. 110033226_ipt_07_磚塊樺木(2x1):151
591. 110033226_ipt_06_磚塊樺木(1x1):145
592. 110033226_ipt_07_磚塊樺木(2x1):152
593. 110033226_ipt_06_磚塊樺木(1x1):146
594. 110033226_ipt_07_磚塊樺木(2x1):153
595. 110033226_ipt_07_磚塊樺木(2x1):154
596. 110033226_ipt_06_磚塊樺木(1x1):147
597. 110033226_ipt_07_磚塊樺木(2x1):155
598. 110033226_ipt_06_磚塊樺木(1x1):148
599. 110033226_ipt_08_平滑面(3x1):17 — 貼合:198, 貼合:278
600. 110033226_ipt_06_磚塊樺木(1x1):149
601. 110033226_ipt_07_磚塊樺木(2x1):156
602. 110033226_ipt_06_磚塊樺木(1x1):150
603. 110033226_ipt_07_磚塊樺木(2x1):157
604. 110033226_ipt_06_磚塊樺木(1x1):151
605. 110033226_ipt_07_磚塊樺木(2x1):158
606. 110033226_ipt_06_磚塊樺木(1x1):152
607. 110033226_ipt_07_磚塊樺木(2x1):159
608. 110033226_ipt_06_磚塊樺木(1x1):153
609. 110033226_ipt_07_磚塊樺木(2x1):160
610. 110033226_ipt_07_磚塊樺木(2x1):161
611. 110033226_ipt_06_磚塊樺木(1x1):154
612. 110033226_ipt_07_磚塊樺木(2x1):162
613. 110033226_ipt_06_磚塊樺木(1x1):155
614. 110033226_ipt_08_平滑面(3x1):18 — 貼合:217, 貼合:218, 貼合:219, 貼合:220, 貼合:221
615. 110033226_ipt_07_磚塊樺木(2x1):24 — 貼合:51, 貼合:52, 貼合:53
616. 110033226_ipt_06_磚塊樺木(1x1):21 — 貼合:56, 貼合:57
617. 110033226_ipt_07_磚塊樺木(2x1):37
618. 110033226_ipt_06_磚塊樺木(1x1):36
619. 110033226_ipt_07_磚塊樺木(2x1):38
620. 110033226_ipt_06_磚塊樺木(1x1):37
621. 110033226_ipt_07_磚塊樺木(2x1):39
622. 110033226_ipt_06_磚塊樺木(1x1):38
623. 110033226_ipt_07_磚塊樺木(2x1):40
624. 110033226_ipt_06_磚塊樺木(1x1):39
625. 110033226_ipt_07_磚塊樺木(2x1):41
626. 110033226_ipt_06_磚塊樺木(1x1):40
627. 110033226_ipt_07_磚塊樺木(2x1):163
628. 110033226_ipt_06_磚塊樺木(1x1):156
629. 110033226_ipt_07_磚塊樺木(2x1):164
630. 110033226_ipt_06_磚塊樺木(1x1):157
631. 110033226_ipt_07_磚塊樺木(2x1):165
632. 110033226_ipt_06_磚塊樺木(1x1):158
633. 110033226_ipt_07_磚塊樺木(2x1):166
634. 110033226_ipt_06_磚塊樺木(1x1):159
635. 110033226_ipt_07_磚塊樺木(2x1):167
636. 110033226_ipt_06_磚塊樺木(1x1):160
637. 110033226_ipt_07_磚塊樺木(2x1):168
638. 110033226_ipt_06_磚塊樺木(1x1):161
639. 110033226_ipt_11_樓梯支架:1 — 貼合:174, 貼合:175, 貼合:176, 貼合:177, 貼合:179
640. 110033226_ipt_11_樓梯支架:3 — 貼合:190
641. 110033226_ipt_11_樓梯支架:4 — 貼合:183, 貼合:188
642. 110033226_ipt_11_樓梯支架:5 — 貼合:182, 貼合:187
643. 110033226_ipt_11_樓梯支架:6 — 貼合:181, 貼合:184, 貼合:422, 貼合:423
644. 110033226_ipt_11_樓梯支架:7 — 貼合:178
645. 110033226_ipt_11_樓梯支架:8 — 貼合:180, 貼合:191
646. 110033226_ipt_11_樓梯支架:9 — 貼合:189
647. 110033226_ipt_11_樓梯支架:10 — 貼合:186
648. 110033226_ipt_11_樓梯支架:11 — 貼合:185, 貼合:421
649. 110033226_ipt_02_草地一:1 — 貼合:298, 貼合:299, 貼合:300, 貼合:324
650. 110033226_ipt_13_草地二:3 — 貼合:301, 貼合:302, 貼合:303
651. 110033226_ipt_02_草地一:4
652. 110033226_ipt_13_草地二:12
653. 110033226_ipt_02_草地一:5 — 貼合:374, 貼合:375, 貼合:376
654. 110033226_ipt_13_草地二:13 — 貼合:371, 貼合:372, 貼合:373
655. 110033226_ipt_02_草地一:2 — 貼合:371, 貼合:372, 貼合:373
656. 110033226_ipt_13_草地二:28 — 貼合:374, 貼合:375, 貼合:376
657. 110033226_ipt_02_草地一:6
658. 110033226_ipt_13_草地二:29
659. 110033226_ipt_02_草地一:7
660. 110033226_ipt_13_草地二:30
661. 110033226_ipt_02_草地一:8
662. 110033226_ipt_13_草地二:31
663. 110033226_ipt_02_草地一:9
664. 110033226_ipt_13_草地二:32
665. 110033226_ipt_02_草地一:10
666. 110033226_ipt_13_草地二:33
667. 110033226_ipt_02_草地一:11
668. 110033226_ipt_13_草地二:34
669. 110033226_ipt_02_草地一:12
670. 110033226_ipt_13_草地二:35
671. 110033226_ipt_02_草地一:13
672. 110033226_ipt_13_草地二:36 — 貼合:377, 貼合:378, 貼合:379, 貼合:380, 貼合:381, 貼合:382
673. 110033226_ipt_10_木板條:9 — 貼合:403, 貼合:404, 貼合:405
674. 110033226_ipt_10_木板條:11 — 貼合:406, 貼合:418
675. 110033226_ipt_10_木板條:12 — 貼合:413, 貼合:417
676. 110033226_ipt_10_木板條:13
677. 110033226_ipt_10_木板條:14
678. 110033226_ipt_10_木板條:15 — 貼合:411, 貼合:412
679. 110033226_ipt_10_木板條:16
680. 110033226_ipt_10_木板條:17 — 貼合:407, 貼合:414
681. 110033226_ipt_10_木板條:18 — 貼合:416
682. 110033226_ipt_10_木板條:20
683. 110033226_ipt_10_木板條:21
684. 110033226_ipt_10_木板條:22
685. 110033226_ipt_10_木板條:23
686. 110033226_ipt_10_木板條:24
687. 110033226_ipt_10_木板條:25
688. 110033226_ipt_10_木板條:26
689. 110033226_ipt_10_木板條:27
690. 110033226_ipt_10_木板條:28
691. 110033226_ipt_10_木板條:8 — 貼合:409, 貼合:410
692. 110033226_ipt_10_木板條:19
693. 110033226_ipt_10_木板條:29 — 貼合:419, 貼合:420
694. 110033226_ipt_10_木板條:30
## Component patterns: (3 elements, first: 110033226_ipt_07_磚塊樺木(2x1):1 + 110033226_ipt_06_磚塊樺木(1x1):1), (6 elements, first: 110033226_ipt_06_磚塊樺木(1x1):2 + 110033226_ipt_07_磚塊樺木(2x1):2), (6 elements, first: 110033226_ipt_07_磚塊樺木(2x1):10 + 110033226_ipt_06_磚塊樺木(1x1):10), (3 elements, first: 110033226_ipt_06_磚塊樺木(1x1):17 + 110033226_ipt_07_磚塊樺木(2x1):18), (6 elements, first: 110033226_ipt_07_磚塊樺木(2x1):21 + 110033226_ipt_06_磚塊樺木(1x1):25), (6 elements, first: 110033226_ipt_06_磚塊樺木(1x1):20 + 110033226_ipt_07_磚塊樺木(2x1):22), (6 elements, first: 110033226_ipt_06_磚塊樺木(1x1):43 + 110033226_ipt_07_磚塊樺木(2x1):46), (6 elements, first: 110033226_ipt_07_磚塊樺木(2x1):44 + 110033226_ipt_06_磚塊樺木(1x1):42), (2 elements, first: 110033226_ipt_06_磚塊樺木(1x1):23 + 110033226_ipt_07_磚塊樺木(2x1):26), (2 elements, first: 110033226_ipt_07_磚塊樺木(2x1):52 + 110033226_ipt_06_磚塊樺木(1x1):45 + 110033226_ipt_06_磚塊樺木(1x1):47 + 110033226_ipt_07_磚塊樺木(2x1):51 + 110033226_ipt_07_磚塊樺木(2x1):47 + 110033226_ipt_06_磚塊樺木(1x1):46), (2 elements, first: 110033226_ipt_07_磚塊樺木(2x1):75 + 110033226_ipt_07_磚塊樺木(2x1):78 + 110033226_ipt_07_磚塊樺木(2x1):73 + 110033226_ipt_07_磚塊樺木(2x1):72), (3 elements, first: 110033226_ipt_07_磚塊樺木(2x1):74 + 110033226_ipt_06_磚塊樺木(1x1):71), (3 elements, first: 110033226_ipt_08_平滑面(3x1):2), (2 elements), (2 elements), (2 elements), (11 elements, first: 110033226_ipt_07_磚塊樺木(2x1):17 + 110033226_ipt_06_磚塊樺木(1x1):16 + 110033226_ipt_07_磚塊樺木(2x1):16), (9 elements, first: 110033226_ipt_08_平滑面(3x1):1), (6 elements, first: 110033226_ipt_08_平滑面(3x1):4), (10 elements, first: 110033226_ipt_07_磚塊樺木(2x1):76 + 110033226_ipt_06_磚塊樺木(1x1):73 + 110033226_ipt_06_磚塊樺木(1x1):66 + 110033226_ipt_07_磚塊樺木(2x1):69), (3 elements, first: 110033226_ipt_07_磚塊樺木(2x1):68 + 110033226_ipt_06_磚塊樺木(1x1):75), (15 elements, first: 110033226_ipt_06_磚塊樺木(1x1):68 + 110033226_ipt_07_磚塊樺木(2x1):210 + 110033226_ipt_06_磚塊樺木(1x1):192 + 110033226_ipt_07_磚塊樺木(2x1):209), (9 elements, first: 110033226_ipt_06_磚塊樺木(1x1):222 + 110033226_ipt_07_磚塊樺木(2x1):239 + 110033226_ipt_06_磚塊樺木(1x1):221 + 110033226_ipt_07_磚塊樺木(2x1):240), (3 elements, first: 110033226_ipt_07_磚塊樺木(2x1):259 + 110033226_ipt_06_磚塊樺木(1x1):242 + 110033226_ipt_07_磚塊樺木(2x1):258 + 110033226_ipt_06_磚塊樺木(1x1):241), (10 elements, first: 110033226_ipt_07_磚塊樺木(2x1):265 + 110033226_ipt_07_磚塊樺木(2x1):266 + 110033226_ipt_06_磚塊樺木(1x1):248 + 110033226_ipt_06_磚塊樺木(1x1):247), (10 elements, first: 110033226_ipt_06_磚塊樺木(1x1):268), (2 elements, first: 110033226_ipt_08_平滑面(3x1):33), (5 elements, first: 110033226_ipt_13_草地二:1), (5 elements, first: 110033226_ipt_13_草地二:2), (5 elements, first: 110033226_ipt_13_草地二:14), (5 elements, first: 110033226_ipt_13_草地二:19), (2 elements), (12 elements, first: 110033226_ipt_14_草地三:19 + 110033226_ipt_14_草地三:18), (4 elements, first: 110033226_ipt_08_平滑面(3x1):37), (2 elements), (2 elements, first: 110033226_ipt_24_直條(3x1):3 + 110033226_ipt_24_直條(3x1):2), (4 elements, first: 110033226_ipt_10_木板條:31), (2 elements, first: 110033226_ipt_10_木板條:35), (6 elements, first: 110033226_ipt_06_磚塊樺木(1x1):44 + 110033226_ipt_07_磚塊樺木(2x1):43 + 110033226_ipt_06_磚塊樺木(1x1):51 + 110033226_ipt_07_磚塊樺木(2x1):49 + 110033226_ipt_06_磚塊樺木(1x1):48 + 110033226_ipt_07_磚塊樺木(2x1):45 + 110033226_ipt_06_磚塊樺木(1x1):74 + 110033226_ipt_07_磚塊樺木(2x1):79 + 110033226_ipt_06_磚塊樺木(1x1):76 + 110033226_ipt_07_磚塊樺木(2x1):70 + 110033226_ipt_07_磚塊樺木(2x1):67 + 110033226_ipt_06_磚塊樺木(1x1):70 + 110033226_ipt_07_磚塊樺木(2x1):71 + 110033226_ipt_06_磚塊樺木(1x1):69 + 110033226_ipt_08_平滑面(3x1):5), 元件陣列 15:2 (6 elements), (6 elements, first: 110033226_ipt_07_磚塊樺木(2x1):24 + 110033226_ipt_06_磚塊樺木(1x1):21), 元件陣列 7:2 (6 elements), (5 elements, first: 110033226_ipt_11_樓梯支架:1), 元件陣列 19:2 (5 elements), (3 elements, first: 110033226_ipt_02_草地一:1 + 110033226_ipt_13_草地二:3), (3 elements, first: 110033226_ipt_02_草地一:2 + 110033226_ipt_13_草地二:28), 元件陣列 35:2 (3 elements), 元件陣列 38:2 (3 elements), (9 elements, first: 110033226_ipt_10_木板條:9), 元件陣列 42:2 (9 elements), (2 elements, first: 110033226_ipt_10_木板條:8), 元件陣列 44:2 (2 elements)
## Relationships (412: Mate 407, Symmetry 4, Angle 1)
- 貼合:1 [Mate]: 110033226_ipt_05_房子底座:1
- 貼合:2 [Mate]: 110033226_ipt_05_房子底座:1
- 貼合:3 [Mate]: 110033226_ipt_05_房子底座:1
- 貼合:4 [Mate]: 110033226_ipt_05_房子底座:1 ↔ 110033226_ipt_07_磚塊樺木(2x1):1
- 貼合:6 [Mate]: 110033226_ipt_05_房子底座:1 ↔ 110033226_ipt_06_磚塊樺木(1x1):1
- 貼合:8 [Mate]: 110033226_ipt_05_房子底座:1 ↔ 110033226_ipt_07_磚塊樺木(2x1):1
- 貼合:9 [Mate]: 110033226_ipt_05_房子底座:1 ↔ 110033226_ipt_06_磚塊樺木(1x1):1
- 貼合:10 [Mate]: 110033226_ipt_05_房子底座:1 ↔ 110033226_ipt_07_磚塊樺木(2x1):1
- 貼合:11 [Mate]: 110033226_ipt_05_房子底座:1 ↔ 110033226_ipt_06_磚塊樺木(1x1):2
- 貼合:12 [Mate]: 110033226_ipt_05_房子底座:1 ↔ 110033226_ipt_07_磚塊樺木(2x1):2
- 貼合:13 [Mate]: 110033226_ipt_05_房子底座:1 ↔ 110033226_ipt_06_磚塊樺木(1x1):2
- 貼合:14 [Mate]: 110033226_ipt_05_房子底座:1 ↔ 110033226_ipt_07_磚塊樺木(2x1):2
- 貼合:15 [Mate]: 110033226_ipt_05_房子底座:1 ↔ 110033226_ipt_07_磚塊樺木(2x1):2
- 貼合:16 [Mate]: 110033226_ipt_05_房子底座:1 ↔ 110033226_ipt_06_磚塊樺木(1x1):10
- 貼合:17 [Mate]: 110033226_ipt_05_房子底座:1 ↔ 110033226_ipt_07_磚塊樺木(2x1):10
- 貼合:18 [Mate]: 110033226_ipt_05_房子底座:1 ↔ 110033226_ipt_07_磚塊樺木(2x1):10
- 貼合:19 [Mate]: 110033226_ipt_05_房子底座:1 ↔ 110033226_ipt_07_磚塊樺木(2x1):10
- 貼合:20 [Mate]: 110033226_ipt_05_房子底座:1 ↔ 110033226_ipt_06_磚塊樺木(1x1):10
- 貼合:21 [Mate]: 110033226_ipt_05_房子底座:1 ↔ 110033226_ipt_07_磚塊樺木(2x1):16
- 貼合:22 [Mate]: 110033226_ipt_05_房子底座:1 ↔ 110033226_ipt_06_磚塊樺木(1x1):16
- 貼合:23 [Mate]: 110033226_ipt_05_房子底座:1 ↔ 110033226_ipt_07_磚塊樺木(2x1):17
- 貼合:24 [Mate]: 110033226_ipt_05_房子底座:1 ↔ 110033226_ipt_06_磚塊樺木(1x1):16
- 貼合:25 [Mate]: 110033226_ipt_05_房子底座:1 ↔ 110033226_ipt_07_磚塊樺木(2x1):16
- 貼合:26 [Mate]: 110033226_ipt_05_房子底座:1 ↔ 110033226_ipt_07_磚塊樺木(2x1):16
- 貼合:27 [Mate]: 110033226_ipt_05_房子底座:1 ↔ 110033226_ipt_07_磚塊樺木(2x1):17
- 貼合:28 [Mate]: 110033226_ipt_05_房子底座:1 ↔ 110033226_ipt_07_磚塊樺木(2x1):17
- 貼合:29 [Mate]: 110033226_ipt_07_磚塊樺木(2x1):1 ↔ 110033226_ipt_07_磚塊樺木(2x1):18
- 貼合:30 [Mate]: 110033226_ipt_07_磚塊樺木(2x1):1 ↔ 110033226_ipt_06_磚塊樺木(1x1):17
- 貼合:31 [Mate]: 110033226_ipt_07_磚塊樺木(2x1):1 ↔ 110033226_ipt_06_磚塊樺木(1x1):17